# Autodesk Inventor assembly: Full Assembly
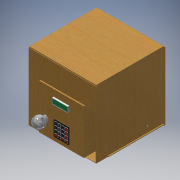
[picture p0: Inventor's stored thumbnail of the model, 180x180]
Saved by Autodesk Inventor 2019 (Build 230136000, 136)
## iProperties
Created: 2018-06-23
Part Number: Full Assembly
Document SubType Name: Assembly
Designer: Akshay
Author: Akshay
## Documents named in this file (15)
- D:\Electronic Safe\CAD\Full Assembly.iam
- D:\Electronic Safe\CAD\door back.ipt
- D:\Electronic Safe\CAD\door right, left, top, bottom.ipt
- D:\Electronic Safe\CAD\front door.ipt
- D:\Electronic Safe\CAD\inge.iam
- D:\Electronic Safe\CAD\keypad.ipt
- D:\Electronic Safe\CAD\knob.ipt
- D:\Electronic Safe\CAD\LCD.ipt
- D:\Electronic Safe\CAD\top,back,left,bottom.ipt
- D:\Electronic Safe\CAD\bl3.ipt
- D:\Electronic Safe\CAD\Pillar front.ipt
- D:\Electronic Safe\CAD\front door cover 3.ipt
- D:\Electronic Safe\CAD\hinge support.ipt
- D:\Electronic Safe\CAD\hinge adjustment.ipt
- D:\Electronic Safe\CAD\right 2.ipt
## Components (19 placed, 14 different names)
1. inge:1 [sub-assembly] — Mate:29, Mate:34, Mate:36
2. top,back,left,bottom:2 — Mate:1, Flush:2, Flush:3, Flush:7, Mate:24, Mate:26, Mate:32, Flush:41, Flush:43
3. top,back,left,bottom:3 — Mate:1, Flush:2, Flush:3, Mate:10, Mate:23, Flush:37, Flush:42
4. top,back,left,bottom:4 — Mate:22
5. bl3:1 — Mate:10, Flush:7, Mate:28, Mate:33
6. door back:1 — Mate:17, Flush:35, Flush:36, Mate:36
7. keypad:1 — Mate:18, Mate:19, Mate:20
8. knob:1 — Mate:21, Rigid:1
9. LCD:1 — Mate:11, Mate:12, Mate:13
10. front door:1 — Mate:11, Mate:12, Mate:13, Mate:14, Flush:26, Flush:27, Mate:15, Flush:28, Flush:29, Flush:30, Flush:32, Mate:16, Mate:18, Mate:19, Mate:20, Mate:21, Rigid:1
11. door right, left, top, bottom:4 — Mate:15, Flush:28, Flush:29, Flush:31, Flush:34, Flush:36
12. door right, left, top, bottom:5 — Flush:30, Flush:31, Flush:32, Flush:35
13. door right, left, top, bottom:6 — Mate:16, Flush:33, Flush:34
14. door right, left, top, bottom:7 — Mate:14, Flush:26, Flush:27, Flush:33, Mate:17, Rotation/Translation:1
15. Pillar front:1 — Mate:22, Mate:23, Flush:37, Mate:37
16. hinge support:1 — Mate:24, Flush:38, Rotation/Translation:1, Mate:29, Mate:34, Mate:35
17. hinge adjustment:1 — Mate:26, Mate:28, Flush:38
18. right 2:1 — Mate:32, Mate:33, Mate:35, Flush:41
19. front door cover 3:1 — Mate:37, Flush:42, Flush:43
## Relationships (46: Mate 25, Flush 19, WeldJoint 1, RelateRotateTranslate 1)
- Mate:1: top,back,left,bottom:2 ↔ top,back,left,bottom:3
- Flush:2: top,back,left,bottom:2 ↔ top,back,left,bottom:3
- Flush:3: top,back,left,bottom:2 ↔ top,back,left,bottom:3
- Mate:10: top,back,left,bottom:3 ↔ bl3:1
- Flush:7: top,back,left,bottom:2 ↔ bl3:1
- Mate:11: LCD:1 ↔ front door:1
- Mate:12: LCD:1 ↔ front door:1
- Mate:13: LCD:1 ↔ front door:1
- Mate:14: front door:1 ↔ door right, left, top, bottom:7
- Flush:26: front door:1 ↔ door right, left, top, bottom:7
- Flush:27: front door:1 ↔ door right, left, top, bottom:7
- Mate:15: front door:1 ↔ door right, left, top, bottom:4
- Flush:28: front door:1 ↔ door right, left, top, bottom:4
- Flush:29: front door:1 ↔ door right, left, top, bottom:4
- Flush:30: front door:1 ↔ door right, left, top, bottom:5
- Flush:31: door right, left, top, bottom:4 ↔ door right, left, top, bottom:5
- Flush:32: front door:1 ↔ door right, left, top, bottom:5
- Mate:16: front door:1 ↔ door right, left, top, bottom:6
- Flush:33: door right, left, top, bottom:6 ↔ door right, left, top, bottom:7
- Flush:34: door right, left, top, bottom:4 ↔ door right, left, top, bottom:6
- Mate:17: door back:1 ↔ door right, left, top, bottom:7
- Flush:35: door back:1 ↔ door right, left, top, bottom:5
- Flush:36: door back:1 ↔ door right, left, top, bottom:4
- Mate:18: keypad:1 ↔ front door:1
- Mate:19: keypad:1 ↔ front door:1
- Mate:20: keypad:1 ↔ front door:1
- Mate:21: knob:1 ↔ front door:1
- Rigid:1 [WeldJoint]: knob:1 ↔ front door:1
- Mate:22: top,back,left,bottom:4 ↔ Pillar front:1
- Mate:23: top,back,left,bottom:3 ↔ Pillar front:1
- Flush:37: top,back,left,bottom:3 ↔ Pillar front:1
- Mate:24: top,back,left,bottom:2 ↔ hinge support:1
- Mate:26: top,back,left,bottom:2 ↔ hinge adjustment:1
- Mate:28: bl3:1 ↔ hinge adjustment:1
- Flush:38: hinge support:1 ↔ hinge adjustment:1
- Rotation/Translation:1 [RelateRotateTranslate] (25.4 mm): door right, left, top, bottom:7 ↔ hinge support:1
- Mate:29: inge:1 ↔ hinge support:1
- Mate:32: top,back,left,bottom:2 ↔ right 2:1
- Mate:33: bl3:1 ↔ right 2:1
- Mate:34: inge:1 ↔ hinge support:1
- Mate:35: hinge support:1 ↔ right 2:1
- Flush:41: top,back,left,bottom:2 ↔ right 2:1
- Mate:36: inge:1 ↔ door back:1
- Mate:37: Pillar front:1 ↔ front door cover 3:1
- Flush:42: top,back,left,bottom:3 ↔ front door cover 3:1
- Flush:43: top,back,left,bottom:2 ↔ front door cover 3:1
